# Autodesk Inventor assembly: non integrated hatch
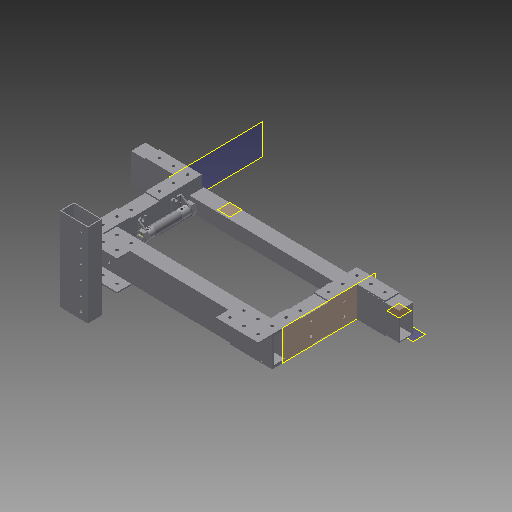
[picture p0: Inventor's stored thumbnail of the model, 512x512]
Saved by Autodesk Inventor 2018.3 (Build 223284000, 284)
## iProperties
Created: 2019-01-26
Part Number: non integrated hatch
Document SubType Name: Assembly
Designer: s-4008082
Author: s-4008082
## Documents named in this file (8)
- C:\Users\Refraction\Documents\GitHub\2019CAD\new Hatch design but everythig is broke\non integrated hatch.iam
- C:\Users\Refraction\Documents\GitHub\2019CAD\new Hatch design but everythig is broke\left arm.ipt
- C:\Users\Refraction\Documents\GitHub\2019CAD\new Hatch design but everythig is broke\push bar.ipt
- C:\Users\Refraction\Documents\GitHub\2019CAD\new Hatch design but everythig is broke\PARTserver02019011803125824465437192d056f\AIS2018\021-DXP(F,D-770).iam
- C:\Users\Refraction\Documents\GitHub\2019CAD\new Hatch design but everythig is broke\Bracing 3x3.ipt
- C:\Users\Refraction\Documents\GitHub\2019CAD\new Hatch design but everythig is broke\ATACHMENT BAR.ipt
- C:\Users\Refraction\Documents\GitHub\2019CAD\new Hatch design but everythig is broke\Mounting part.ipt
- C:\Users\Refraction\Documents\GitHub\2019CAD\new Hatch design but everythig is broke\bar thing.ipt
## Components (17 placed, 7 different names)
1. left arm:1 — Flush:23, Flush:28, Flush:29, Flush:32, Mate:37, Flush:34, Mate:38, Flush:35, Mate:41, Mate:42, Flush:37, Mate:47
2. push bar:1
3. 021-DXP(F,D-770):1 [sub-assembly] — Mate:41, Mate:42, Flush:37, Mate:47, Flush:43, Flush:46, Flush:47
4. 021-DXP(F,D-770):2 [sub-assembly] — Flush:43, Mate:50, Flush:46, Flush:47
5. Bracing 3x3:1 — Flush:28, Flush:29, Flush:30, Mate:38
6. Bracing 3x3:2 — Flush:22, Flush:31, Flush:32, Flush:33, Mate:37
7. Bracing 3x3:3 — Mate:33
8. Bracing 3x3:4 — Mate:30, Flush:24
9. Bracing 3x3:5 — Mate:36
10. Bracing 3x3:6
11. Bracing 3x3:7 — Flush:45
12. Bracing 3x3:8 — Flush:36
13. ATACHMENT BAR:1 — Mate:36, Flush:35, Flush:36, Mate:43, Mate:44, Mate:48, Mate:49, Flush:44
14. Mounting part:1 — Mate:43, Mate:44, Mate:48
15. bar thing:1 — Flush:22, Flush:23, Flush:30, Flush:31, Flush:33, Flush:34
16. bar thing:2 — Mate:30, Flush:24, Mate:33
17. left arm:2 — Mate:49, Flush:44, Flush:45, Mate:50
## Relationships (38: Flush 19, Mate 19)
- [Flush]: left arm:1 ↔ Bracing 3x3:2
- [Mate] (2.54 mm): push bar:1 ↔ 021-DXP(F,D-770):2
- [Mate]: push bar:1 ↔ 021-DXP(F,D-770):2
- [Mate] (2.54 mm): push bar:1 ↔ 021-DXP(F,D-770):1
- [Mate]: push bar:1 ↔ 021-DXP(F,D-770):1
- [Mate]: left arm:1 ↔ Bracing 3x3:5
- [Mate]: Bracing 3x3:7 ↔ ATACHMENT BAR:1
- Flush:22: Bracing 3x3:2 ↔ bar thing:1
- Flush:23: left arm:1 ↔ bar thing:1
- Mate:30: Bracing 3x3:4 ↔ bar thing:2
- Flush:24: Bracing 3x3:4 ↔ bar thing:2
- Mate:33: Bracing 3x3:3 ↔ bar thing:2
- Mate:36: Bracing 3x3:5 ↔ ATACHMENT BAR:1
- Flush:28: left arm:1 ↔ Bracing 3x3:1
- Flush:29: left arm:1 ↔ Bracing 3x3:1
- Flush:30: Bracing 3x3:1 ↔ bar thing:1
- Flush:31: Bracing 3x3:2 ↔ bar thing:1
- Flush:32: left arm:1 ↔ Bracing 3x3:2
- Flush:33: Bracing 3x3:2 ↔ bar thing:1
- Mate:37: left arm:1 ↔ Bracing 3x3:2
- Flush:34: left arm:1 ↔ bar thing:1
- Mate:38: left arm:1 ↔ Bracing 3x3:1
- Flush:35: left arm:1 ↔ ATACHMENT BAR:1
- Flush:36: Bracing 3x3:8 ↔ ATACHMENT BAR:1
- Mate:41: left arm:1 ↔ 021-DXP(F,D-770):1
- Mate:42: left arm:1 ↔ 021-DXP(F,D-770):1
- Flush:37 (38.1 mm): left arm:1 ↔ 021-DXP(F,D-770):1
- Mate:43: ATACHMENT BAR:1 ↔ Mounting part:1
- Mate:44 (-101.6 mm): ATACHMENT BAR:1 ↔ Mounting part:1
- Mate:47: left arm:1 ↔ 021-DXP(F,D-770):1
- Flush:43: 021-DXP(F,D-770):1 ↔ 021-DXP(F,D-770):2
- Mate:48: ATACHMENT BAR:1 ↔ Mounting part:1
- Mate:49: ATACHMENT BAR:1 ↔ left arm:2
- Flush:44: ATACHMENT BAR:1 ↔ left arm:2
- Flush:45: Bracing 3x3:7 ↔ left arm:2
- Mate:50: 021-DXP(F,D-770):2 ↔ left arm:2
- Flush:46: 021-DXP(F,D-770):1 ↔ 021-DXP(F,D-770):2
- Flush:47: 021-DXP(F,D-770):1 ↔ 021-DXP(F,D-770):2
